# Autodesk Inventor assembly: Assembly1
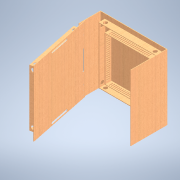
[picture p0: Inventor's stored thumbnail of the model, 180x180]
Saved by Autodesk Inventor 2020 (Build 240168000, 168)
## iProperties
Created: 2020-05-02
Part Number: Assembly1
Document SubType Name: Assembly
Designer: galaxy
Author: galaxy
## Documents named in this file (5)
- C:\Users\galaxy\Desktop\control box\Assembly1.iam
- C:\Users\galaxy\Desktop\control box\back.ipt
- C:\Users\galaxy\Desktop\control box\left_joint.iam
- C:\Users\galaxy\Desktop\control box\middle_joints.iam
- C:\Users\galaxy\Desktop\control box\rightside.ipt
## Components (4 placed, 4 different names)
1. back:1 — Mate:1, Mate:2, Mate:3, Mate:4
2. left_joint:1 [sub-assembly] — Mate:1, Mate:2, Insert:1
3. middle_joints:1 [sub-assembly] — Insert:1
4. rightside:1 — Mate:3, Mate:4
## Relationships (5: Mate 4, Insert 1)
- Mate:1: back:1 ↔ left_joint:1
- Mate:2: back:1 ↔ left_joint:1
- Insert:1: left_joint:1 ↔ middle_joints:1
- Mate:3: back:1 ↔ rightside:1
- Mate:4: back:1 ↔ rightside:1
